# Autodesk Inventor assembly: Lift.02.00.00.00
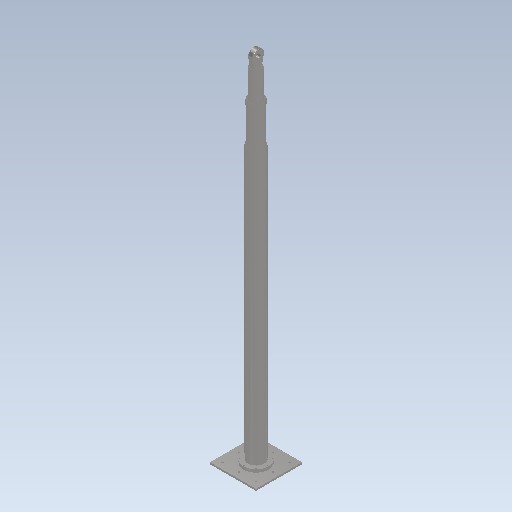
[picture p0: Inventor's stored thumbnail of the model, 512x512]
Saved by Autodesk Inventor 2021 (Build 250183000, 183)
## iProperties
Created: 2020-09-20
Part Number: Lift.02.00.00.00
Document SubType Name: Assembly
Designer: Kostya
Author: Kostya
## Documents named in this file (7)
- C:\Lift\Lift.02.00.00.00.iam
- C:\Lift\Lift.02.00.00.06.ipt
- C:\Lift\Lift.02.00.00.05.ipt
- C:\Lift\Lift.02.00.00.04.ipt
- C:\Lift\Lift.02.00.00.03.ipt
- C:\Lift\Lift.02.00.00.02.ipt
- C:\Lift\Lift.02.00.00.01.ipt
## Components (6 placed, 6 different names)
1. Lift.02.00.00.06:1 — Совмещение:1, Заподлицо:1, Совмещение:3, Совмещение:4, Заподлицо:2, Совмещение:5
2. Lift.02.00.00.05:1 — Совмещение:9, Совмещение:10, Совмещение:14
3. Lift.02.00.00.04:1 — Совмещение:8, Совмещение:9, Совмещение:10, Совмещение:11
4. Lift.02.00.00.03:1 — Совмещение:7, Совмещение:8, Совмещение:11, Совмещение:12
5. Lift.02.00.00.02:1 — Совмещение:6, Совмещение:7, Совмещение:12, Совмещение:13
6. Lift.02.00.00.01:1 — Совмещение:3, Совмещение:4, Заподлицо:2, Совмещение:6, Совмещение:13
## Relationships (15: Mate 13, Flush 2)
- Совмещение:1 [Mate]: Lift.02.00.00.06:1
- Заподлицо:1 [Flush]: Lift.02.00.00.06:1
- Совмещение:3 [Mate]: Lift.02.00.00.06:1 ↔ Lift.02.00.00.01:1
- Совмещение:4 [Mate]: Lift.02.00.00.06:1 ↔ Lift.02.00.00.01:1
- Заподлицо:2 [Flush]: Lift.02.00.00.06:1 ↔ Lift.02.00.00.01:1
- Совмещение:5 [Mate]: Lift.02.00.00.06:1
- Совмещение:6 [Mate]: Lift.02.00.00.02:1 ↔ Lift.02.00.00.01:1
- Совмещение:7 [Mate]: Lift.02.00.00.03:1 ↔ Lift.02.00.00.02:1
- Совмещение:8 [Mate]: Lift.02.00.00.04:1 ↔ Lift.02.00.00.03:1
- Совмещение:9 [Mate]: Lift.02.00.00.05:1 ↔ Lift.02.00.00.04:1
- Совмещение:10 [Mate]: Lift.02.00.00.05:1 ↔ Lift.02.00.00.04:1
- Совмещение:11 [Mate]: Lift.02.00.00.04:1 ↔ Lift.02.00.00.03:1
- Совмещение:12 [Mate]: Lift.02.00.00.03:1 ↔ Lift.02.00.00.02:1
- Совмещение:13 [Mate]: Lift.02.00.00.02:1 ↔ Lift.02.00.00.01:1
- Совмещение:14 [Mate]: Lift.02.00.00.05:1
